# Autodesk Inventor assembly: motor with bevel pinion gear
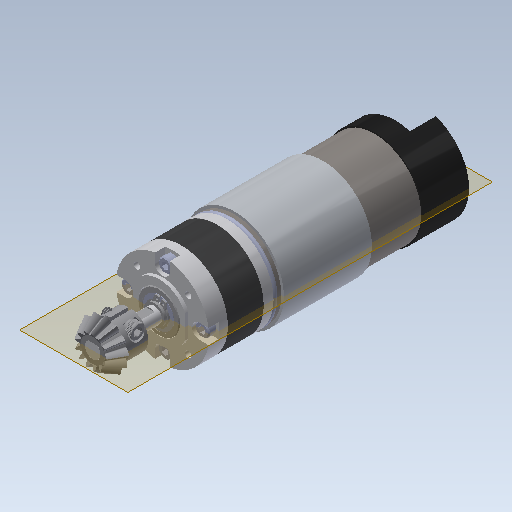
[picture p0: Inventor's stored thumbnail of the model, 512x512]
Saved by Autodesk Inventor 2020 (Build 240168000, 168)
## iProperties
Created: 2019-09-29
Part Number: motor with bevel pinion gear
Document SubType Name: Assembly
Designer: ball
Author: ball
## Documents named in this file (3)
- D:\FTC8863\2019 Robot\Mecanum Drive Train\motor with bevel pinion gear.iam
- D:\FTC8863\Andymark\am-3461a+NeveRest+Orbital+3.7+REV2.ipt
- D:\FTC8863\Actobotics\615 parts\615458 assembly.ipt
## Components (2 placed, 2 different names)
1. am-3461a+NeveRest+Orbital+3.7+REV2:1 — Mate:1, Flush:1, Mate:2, Mate:3
2. 615458 assembly:1 — Mate:1, Flush:1
## Relationships (4: Mate 3, Flush 1)
- Mate:1: am-3461a+NeveRest+Orbital+3.7+REV2:1 ↔ 615458 assembly:1
- Flush:1: am-3461a+NeveRest+Orbital+3.7+REV2:1 ↔ 615458 assembly:1
- Mate:2: am-3461a+NeveRest+Orbital+3.7+REV2:1
- Mate:3: am-3461a+NeveRest+Orbital+3.7+REV2:1
